# Autodesk Inventor assembly: ENSAMBLE_NUEVA_CREMALLERA
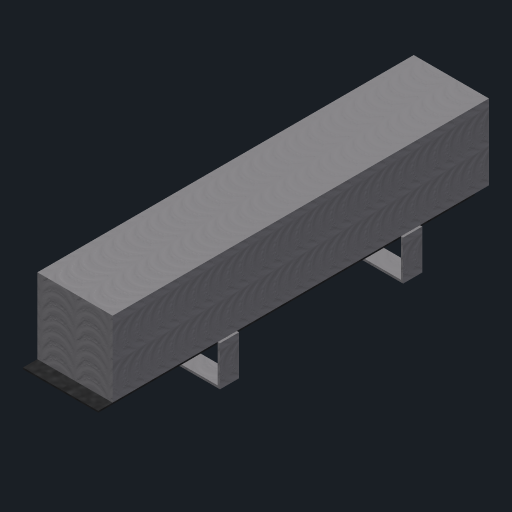
[picture p0: Inventor's stored thumbnail of the model, 512x512]
Saved by Autodesk Inventor 2024.3 (Build 283343000, 343)
## iProperties
Created: 2024-08-24
Part Number: ENSAMBLE_NUEVA_CREMALLERA
Material: Generic
Document SubType Name: Assembly
Designer: Niler
Author: Niler
## Documents named in this file (4)
- C:\Users\Niler\OneDrive\Escritorio\RECICLADOR\RECICLADOR_MODELO_3D\NUEVA CREMALLERA\ENSAMBLE_NUEVA_CREMALLERA.iam
- C:\Users\Niler\OneDrive\Escritorio\RECICLADOR\RECICLADOR_MODELO_3D\NUEVA CREMALLERA\TUBO.ipt
- C:\Users\Niler\OneDrive\Escritorio\RECICLADOR\RECICLADOR_MODELO_3D\NUEVA CREMALLERA\DESLIZANTE.ipt
- C:\Users\Niler\OneDrive\Escritorio\RECICLADOR\RECICLADOR_MODELO_3D\NUEVA CREMALLERA\APOYO_PLETINA.ipt
## Components (4 placed, 3 different names)
1. TUBO:1 — Flush:1, Mate:1, Mate:2, Mate:3, Mate:4, Mate:5
2. DESLIZANTE:1 — Flush:1, Mate:1
3. APOYO_PLETINA:1 — Mate:2, Mate:3
4. APOYO_PLETINA:2 — Mate:4, Mate:5
## Relationships (6: Mate 5, Flush 1)
- Flush:1: TUBO:1 ↔ DESLIZANTE:1
- Mate:1: TUBO:1 ↔ DESLIZANTE:1
- Mate:2: TUBO:1 ↔ APOYO_PLETINA:1
- Mate:3: TUBO:1 ↔ APOYO_PLETINA:1
- Mate:4: TUBO:1 ↔ APOYO_PLETINA:2
- Mate:5: TUBO:1 ↔ APOYO_PLETINA:2
